# Autodesk Inventor assembly: sorterbucket
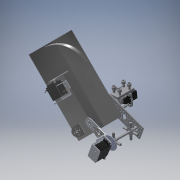
[picture p0: Inventor's stored thumbnail of the model, 180x180]
Saved by Autodesk Inventor 2019 (Build 230136000, 136)
## iProperties
Created: 2018-12-06
Part Number: sorterbucket
Document SubType Name: Assembly
Designer: User
Author: User
## Documents named in this file (13)
- C:\Robotics\CAD\2018-19_CAD\Collection\sorterbucket.iam
- C:\Robotics\CAD\2018-19_CAD\Collection\Sorter.ipt
- C:\Robotics\CAD\COTSParts\Rev\REV-41-1097SmartServo.ipt
- C:\Robotics\CAD\COTSParts\Actobotics\585 parts\585580FlatTriplePatternBracket.ipt
- C:\Robotics\CAD\COTSParts\Tetrix\39274_txm-flat64mmx27mm.ipt
- C:\Robotics\CAD\COTSParts\Tetrix\Tetrix bracket - angle.ipt
- C:\Robotics\CAD\COTSParts\Tetrix\Tetrix servo 180.ipt
- C:\Robotics\CAD\COTSParts\Tetrix\39060_txm-standard servo bracket.ipt
- C:\Robotics\CAD\COTSParts\Actobotics\634 parts\634078.25inDShaft3.5inLong.ipt
- C:\Robotics\CAD\COTSParts\Rev\REV-41-1363ServoHorn.ipt
- C:\Robotics\CAD\2018-19_CAD\Collection\SweeperHub.ipt
- C:\Robotics\CAD\2018-19_CAD\smart servo with servo block.iam
- C:\Robotics\CAD\2018-19_CAD\Collection\20X20 carege assembly.iam
## Components (17 placed, 12 different names)
1. Sorter:1 — Mate:1, Mate:6, Mate:27, Mate:28, Flush:4, Mate:35, Flush:5, Flush:6, Mate:38, Mate:40, Mate:41, Angle:5
2. 585580FlatTriplePatternBracket:1 — Mate:1, Mate:13, Angle:2, Mate:23, Mate:24, Mate:26, Angle:5
3. 39274_txm-flat64mmx27mm:1 — Mate:4, Mate:5, Flush:1, Mate:6, Angle:2
4. Tetrix bracket - angle:1 — Mate:4, Mate:5, Flush:1, Mate:7, Mate:37
5. 39060_txm-standard servo bracket:1 — Mate:7, Mate:14, Mate:15, Mate:16, Mate:37
6. 634078.25inDShaft3.5inLong:1 — Mate:13, Mate:19, Mate:20, Mate:21, Mate:22, Angle:4, Mate:40, Mate:41
7. REV-41-1097SmartServo:1 — Mate:14, Mate:15, Mate:16, Mate:17, Mate:18
8. REV-41-1363ServoHorn:1 — Mate:17, Mate:18, Mate:19, Mate:20
9. SweeperHub:1 — Mate:22, Flush:2
10. SweeperHub:2 — Mate:21, Flush:2, Angle:4
11. smart servo with servo block:1 [sub-assembly] — Mate:23, Mate:24, Mate:25, Flush:3
12. 20X20 carege assembly:1 [sub-assembly] — Mate:25, Mate:26, Flush:3
13. Tetrix servo 180:1 — Mate:27, Mate:29, Mate:30, Angle:3, Mate:33, Mate:34
14. 39060_txm-standard servo bracket:2 — Mate:28, Mate:29, Mate:30, Angle:3, Flush:4
15. 39274_txm-flat64mmx27mm:2 — Mate:33, Mate:34
16. Tetrix bracket - angle:2 — Mate:38, Flush:7, Flush:8
17. Tetrix bracket - angle:3 — Mate:35, Flush:5, Flush:6, Flush:7, Flush:8
## Relationships (42: Mate 30, Flush 8, Angle 4)
- Mate:1: Sorter:1 ↔ 585580FlatTriplePatternBracket:1
- Mate:4: 39274_txm-flat64mmx27mm:1 ↔ Tetrix bracket - angle:1
- Mate:5: 39274_txm-flat64mmx27mm:1 ↔ Tetrix bracket - angle:1
- Flush:1: 39274_txm-flat64mmx27mm:1 ↔ Tetrix bracket - angle:1
- Mate:6: Sorter:1 ↔ 39274_txm-flat64mmx27mm:1
- Mate:7: Tetrix bracket - angle:1 ↔ 39060_txm-standard servo bracket:1
- Mate:13: 585580FlatTriplePatternBracket:1 ↔ 634078.25inDShaft3.5inLong:1
- Mate:14: 39060_txm-standard servo bracket:1 ↔ REV-41-1097SmartServo:1
- Mate:15: 39060_txm-standard servo bracket:1 ↔ REV-41-1097SmartServo:1
- Mate:16: 39060_txm-standard servo bracket:1 ↔ REV-41-1097SmartServo:1
- Mate:17: REV-41-1097SmartServo:1 ↔ REV-41-1363ServoHorn:1
- Mate:18: REV-41-1097SmartServo:1 ↔ REV-41-1363ServoHorn:1
- Mate:19: 634078.25inDShaft3.5inLong:1 ↔ REV-41-1363ServoHorn:1
- Angle:2 (0 deg): 585580FlatTriplePatternBracket:1 ↔ 39274_txm-flat64mmx27mm:1
- Mate:20: 634078.25inDShaft3.5inLong:1 ↔ REV-41-1363ServoHorn:1
- Mate:21: 634078.25inDShaft3.5inLong:1 ↔ SweeperHub:2
- Mate:22: 634078.25inDShaft3.5inLong:1 ↔ SweeperHub:1
- Flush:2: SweeperHub:1 ↔ SweeperHub:2
- Mate:23: 585580FlatTriplePatternBracket:1 ↔ smart servo with servo block:1
- Mate:24: 585580FlatTriplePatternBracket:1 ↔ smart servo with servo block:1
- Mate:25: smart servo with servo block:1 ↔ 20X20 carege assembly:1
- Mate:26 (2.54 mm): 585580FlatTriplePatternBracket:1 ↔ 20X20 carege assembly:1
- Flush:3 (-2.54 mm): smart servo with servo block:1 ↔ 20X20 carege assembly:1
- Mate:27: Sorter:1 ↔ Tetrix servo 180:1
- Mate:28: Sorter:1 ↔ 39060_txm-standard servo bracket:2
- Mate:29: Tetrix servo 180:1 ↔ 39060_txm-standard servo bracket:2
- Mate:30: Tetrix servo 180:1 ↔ 39060_txm-standard servo bracket:2
- Angle:3 (0 deg): Tetrix servo 180:1 ↔ 39060_txm-standard servo bracket:2
- Flush:4: Sorter:1 ↔ 39060_txm-standard servo bracket:2
- Mate:33: Tetrix servo 180:1 ↔ 39274_txm-flat64mmx27mm:2
- Mate:34: Tetrix servo 180:1 ↔ 39274_txm-flat64mmx27mm:2
- Angle:4 (0 deg): 634078.25inDShaft3.5inLong:1 ↔ SweeperHub:2
- Mate:35: Sorter:1 ↔ Tetrix bracket - angle:3
- Flush:5 (-38.1 mm): Sorter:1 ↔ Tetrix bracket - angle:3
- Flush:6 (6.35 mm): Sorter:1 ↔ Tetrix bracket - angle:3
- Mate:37: Tetrix bracket - angle:1 ↔ 39060_txm-standard servo bracket:1
- Mate:38: Sorter:1 ↔ Tetrix bracket - angle:2
- Flush:7: Tetrix bracket - angle:2 ↔ Tetrix bracket - angle:3
- Flush:8: Tetrix bracket - angle:2 ↔ Tetrix bracket - angle:3
- Mate:40 (97.79 mm): Sorter:1 ↔ 634078.25inDShaft3.5inLong:1
- Mate:41 (38.1 mm): Sorter:1 ↔ 634078.25inDShaft3.5inLong:1
- Angle:5 (-25 deg): Sorter:1 ↔ 585580FlatTriplePatternBracket:1
